# Autodesk Inventor assembly: RobotAsem
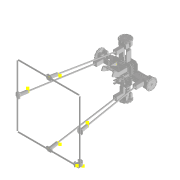
[picture p0: Inventor's stored thumbnail of the model, 180x180]
Saved by Autodesk Inventor 2022 (Build 260153000, 153)
## iProperties
Created: 2022-10-20
Part Number: RobotAsem
Document SubType Name: Assembly
Designer: MVeszpremi
Author: MVeszpremi
## Documents named in this file (20)
- C:\Users\veszp\Dropbox\180DAB CAD\RobotAsem_v2.iam
- C:\Users\veszp\Dropbox\180DAB CAD\RobotBase.ipt
- C:\Users\veszp\Dropbox\180DAB CAD\StepperMotorHolder.ipt
- C:\Users\veszp\Dropbox\180DAB CAD\RobotBaseMotorExt.ipt
- C:\Users\veszp\Dropbox\180DAB CAD\Placeholde_stepperdriverr.ipt
- C:\Users\veszp\Dropbox\180DAB CAD\Wheel.ipt
- C:\Users\veszp\Dropbox\180DAB CAD\RobotBaseMotorExtUpper.ipt
- C:\Users\veszp\Dropbox\180DAB CAD\RaspberryMount.ipt
- C:\Users\veszp\Dropbox\180DAB CAD\RaspberryPiZeroW.ipt
- C:\Users\veszp\Dropbox\180DAB CAD\BatteryMount.ipt
- C:\Users\veszp\Dropbox\180DAB CAD\ExtConnector.ipt
- C:\Users\veszp\Dropbox\180DAB CAD\DriverHolderInside_V2.ipt
- C:\Users\veszp\Dropbox\180DAB CAD\TrayHolder\Shaft_Mount_Lower.ipt
- C:\Users\veszp\Dropbox\180DAB CAD\TrayHolder\Shaft_1.ipt
- C:\Users\veszp\Dropbox\180DAB CAD\TrayHolder\Shaft_Connector_Top.ipt
- C:\Users\veszp\Dropbox\180DAB CAD\TrayHolder\Shaft_2.ipt
- C:\Users\veszp\Dropbox\180DAB CAD\TrayHolder\Shaft_Connector_Top_Corner.ipt
- C:\Users\veszp\Dropbox\180DAB CAD\StereoVisionHolder.iam
- C:\Users\veszp\Dropbox\180DAB CAD\EStopHolder.ipt
- C:\Users\veszp\Dropbox\180DAB CAD\BatteryHolder.ipt
## Components (45 placed, 19 different names)
1. RobotBase:1 — Mate:1, Mate:2, Mate:3, Mate:4, Mate:5, Mate:6, Mate:7, Mate:8, Mate:9, Mate:10, Mate:11, Mate:12, Mate:60, Mate:61, Mate:64, Mate:65, Mate:66
2. RobotBaseMotorExt:1 — Mate:1, Mate:2, Mate:3, Mate:25, Mate:26, Mate:36, Mate:37, Mate:38
3. RobotBaseMotorExt:2 — Mate:4, Mate:5, Mate:6, Mate:27, Mate:28, Mate:29
4. RobotBaseMotorExt:3 — Mate:7, Mate:8, Mate:9, Mate:33, Mate:34, Mate:35, Mate:67
5. RobotBaseMotorExt:4 — Mate:10, Mate:11, Mate:12, Mate:30, Mate:31, Mate:32
6. Placeholde_stepperdriverr:1 — Mate:25, Mate:26
7. StepperMotorHolder:1 — Mate:27, Mate:28, Mate:29, Mate:43
8. StepperMotorHolder:2 — Mate:30, Mate:31, Mate:32, Mate:41, Mate:47, Mate:48, Mate:49
9. StepperMotorHolder:3 — Mate:33, Mate:34, Mate:35, Mate:42, Mate:56
10. StepperMotorHolder:4 — Mate:36, Mate:37, Mate:38, Mate:39, Mate:40
11. Wheel:1 — Mate:39, Mate:40
12. Wheel:2 — Mate:41
13. Wheel:3 — Mate:42, Mate:67
14. Wheel:4 — Mate:43
15. RobotBaseMotorExtUpper:1 — Mate:44, Mate:45, Mate:46, Mate:47, Mate:48, Mate:49, Mate:84, Mate:85, Mate:86
16. RobotBase:2 — Mate:44, Mate:45, Mate:46, Mate:50, Mate:51, Mate:52, Mate:53, Mate:54, Mate:55, Mate:57, Mate:58, Mate:59, Mate:72, Mate:73, Mate:74, Mate:75, Mate:76, Mate:77, Mate:112, Mate:113, Mate:114
17. RobotBaseMotorExtUpper:2 — Mate:50, Mate:51, Mate:52, Mate:81, Mate:82, Mate:83, Mate:115, Mate:116
18. RobotBaseMotorExtUpper:3 — Mate:53, Mate:54, Mate:55, Mate:78, Mate:79, Mate:80, Mate:117, Mate:118, Mate:119
19. RobotBaseMotorExtUpper:4 — Mate:56, Mate:57, Mate:58, Mate:68, Mate:69, Mate:70, Mate:87, Mate:88, Mate:89
20. RaspberryMount:1 — Mate:59, Mate:60, Mate:61, Mate:62, Angle:1, Mate:63
21. RaspberryPiZeroW:1 — Mate:62, Angle:1, Mate:63
22. BatteryMount:1 — Mate:64, Mate:65, Mate:66
23. ExtConnector:1 — Mate:68, Mate:69, Mate:70
24. DriverHolderInside_V2:1 — Mate:72, Mate:73, Mate:74
25. DriverHolderInside_V2:2 — Mate:75, Mate:76, Mate:77
26. Shaft_Mount_Lower:1 — Mate:78, Mate:79, Mate:80, Mate:94, Mate:95
27. Shaft_Mount_Lower:2 — Mate:81, Mate:82, Mate:83, Mate:96, Mate:97
28. Shaft_Mount_Lower:3 — Mate:84, Mate:85, Mate:86, Mate:92, Mate:93
29. Shaft_Mount_Lower:4 — Mate:87, Mate:88, Mate:89, Mate:90, Mate:91
30. Shaft_1:1 — Mate:92, Mate:93, Mate:98, Mate:99
31. Shaft_1:2 — Mate:94, Mate:95, Mate:102, Mate:103
32. Shaft_1:3 — Mate:96, Mate:97, Mate:104, Mate:105
33. Shaft_1:4 — Mate:90, Mate:91, Mate:100, Mate:101
34. Shaft_Connector_Top:1 — Mate:98, Mate:99, Angle:3, Mate:106
35. Shaft_Connector_Top:2 — Mate:100, Mate:101, Angle:2, Mate:109
36. Shaft_Connector_Top:3 — Mate:102, Mate:103, Angle:3, Mate:107
37. Shaft_Connector_Top:4 — Mate:104, Mate:105, Angle:2, Mate:108
38. Shaft_2:1 — Mate:106
39. Shaft_2:2 — Mate:109, Mate:111
40. Shaft_2:3 — Mate:108
41. Shaft_2:4 — Mate:107, Mate:110
42. Shaft_Connector_Top_Corner:1 — Mate:110, Mate:111
43. StereoVisionHolder:1 [sub-assembly] — Mate:112, Mate:113, Mate:114
44. EStopHolder:1 — Mate:115, Mate:116
45. BatteryHolder:1 — Mate:117, Mate:118, Mate:119
## Relationships (109: Mate 106, Angle 3)
- Mate:1: RobotBase:1 ↔ RobotBaseMotorExt:1
- Mate:2: RobotBase:1 ↔ RobotBaseMotorExt:1
- Mate:3: RobotBase:1 ↔ RobotBaseMotorExt:1
- Mate:4: RobotBase:1 ↔ RobotBaseMotorExt:2
- Mate:5: RobotBase:1 ↔ RobotBaseMotorExt:2
- Mate:6: RobotBase:1 ↔ RobotBaseMotorExt:2
- Mate:7: RobotBase:1 ↔ RobotBaseMotorExt:3
- Mate:8: RobotBase:1 ↔ RobotBaseMotorExt:3
- Mate:9: RobotBase:1 ↔ RobotBaseMotorExt:3
- Mate:10: RobotBase:1 ↔ RobotBaseMotorExt:4
- Mate:11: RobotBase:1 ↔ RobotBaseMotorExt:4
- Mate:12: RobotBase:1 ↔ RobotBaseMotorExt:4
- Mate:25: RobotBaseMotorExt:1 ↔ Placeholde_stepperdriverr:1
- Mate:26 (6.5 mm): RobotBaseMotorExt:1 ↔ Placeholde_stepperdriverr:1
- Mate:27: RobotBaseMotorExt:2 ↔ StepperMotorHolder:1
- Mate:28: RobotBaseMotorExt:2 ↔ StepperMotorHolder:1
- Mate:29: RobotBaseMotorExt:2 ↔ StepperMotorHolder:1
- Mate:30: RobotBaseMotorExt:4 ↔ StepperMotorHolder:2
- Mate:31: RobotBaseMotorExt:4 ↔ StepperMotorHolder:2
- Mate:32: RobotBaseMotorExt:4 ↔ StepperMotorHolder:2
- Mate:33: RobotBaseMotorExt:3 ↔ StepperMotorHolder:3
- Mate:34: RobotBaseMotorExt:3 ↔ StepperMotorHolder:3
- Mate:35: RobotBaseMotorExt:3 ↔ StepperMotorHolder:3
- Mate:36: RobotBaseMotorExt:1 ↔ StepperMotorHolder:4
- Mate:37: RobotBaseMotorExt:1 ↔ StepperMotorHolder:4
- Mate:38: RobotBaseMotorExt:1 ↔ StepperMotorHolder:4
- Mate:39: StepperMotorHolder:4 ↔ Wheel:1
- Mate:40 (5.5 mm): StepperMotorHolder:4 ↔ Wheel:1
- Mate:41: StepperMotorHolder:2 ↔ Wheel:2
- Mate:42: StepperMotorHolder:3 ↔ Wheel:3
- Mate:43: StepperMotorHolder:1 ↔ Wheel:4
- Mate:44: RobotBaseMotorExtUpper:1 ↔ RobotBase:2
- Mate:45: RobotBaseMotorExtUpper:1 ↔ RobotBase:2
- Mate:46: RobotBaseMotorExtUpper:1 ↔ RobotBase:2
- Mate:47: StepperMotorHolder:2 ↔ RobotBaseMotorExtUpper:1
- Mate:48: StepperMotorHolder:2 ↔ RobotBaseMotorExtUpper:1
- Mate:49: StepperMotorHolder:2 ↔ RobotBaseMotorExtUpper:1
- Mate:50: RobotBase:2 ↔ RobotBaseMotorExtUpper:2
- Mate:51: RobotBase:2 ↔ RobotBaseMotorExtUpper:2
- Mate:52: RobotBase:2 ↔ RobotBaseMotorExtUpper:2
- Mate:53: RobotBase:2 ↔ RobotBaseMotorExtUpper:3
- Mate:54: RobotBase:2 ↔ RobotBaseMotorExtUpper:3
- Mate:55: RobotBase:2 ↔ RobotBaseMotorExtUpper:3
- Mate:56: StepperMotorHolder:3 ↔ RobotBaseMotorExtUpper:4
- Mate:57: RobotBase:2 ↔ RobotBaseMotorExtUpper:4
- Mate:58: RobotBase:2 ↔ RobotBaseMotorExtUpper:4
- Mate:59: RobotBase:2 ↔ RaspberryMount:1
- Mate:60: RobotBase:1 ↔ RaspberryMount:1
- Mate:61: RobotBase:1 ↔ RaspberryMount:1
- Mate:62: RaspberryMount:1 ↔ RaspberryPiZeroW:1
- Angle:1 (0 deg): RaspberryMount:1 ↔ RaspberryPiZeroW:1
- Mate:63: RaspberryMount:1 ↔ RaspberryPiZeroW:1
- Mate:64: RobotBase:1 ↔ BatteryMount:1
- Mate:65: RobotBase:1 ↔ BatteryMount:1
- Mate:66: RobotBase:1 ↔ BatteryMount:1
- Mate:67 (7.5 mm): RobotBaseMotorExt:3 ↔ Wheel:3
- Mate:68: RobotBaseMotorExtUpper:4 ↔ ExtConnector:1
- Mate:69: RobotBaseMotorExtUpper:4 ↔ ExtConnector:1
- Mate:70: RobotBaseMotorExtUpper:4 ↔ ExtConnector:1
- Mate:72: RobotBase:2 ↔ DriverHolderInside_V2:1
- Mate:73: RobotBase:2 ↔ DriverHolderInside_V2:1
- Mate:74: RobotBase:2 ↔ DriverHolderInside_V2:1
- Mate:75: RobotBase:2 ↔ DriverHolderInside_V2:2
- Mate:76: RobotBase:2 ↔ DriverHolderInside_V2:2
- Mate:77: RobotBase:2 ↔ DriverHolderInside_V2:2
- Mate:78: RobotBaseMotorExtUpper:3 ↔ Shaft_Mount_Lower:1
- Mate:79: RobotBaseMotorExtUpper:3 ↔ Shaft_Mount_Lower:1
- Mate:80: RobotBaseMotorExtUpper:3 ↔ Shaft_Mount_Lower:1
- Mate:81: RobotBaseMotorExtUpper:2 ↔ Shaft_Mount_Lower:2
- Mate:82: RobotBaseMotorExtUpper:2 ↔ Shaft_Mount_Lower:2
- Mate:83: RobotBaseMotorExtUpper:2 ↔ Shaft_Mount_Lower:2
- Mate:84: RobotBaseMotorExtUpper:1 ↔ Shaft_Mount_Lower:3
- Mate:85: RobotBaseMotorExtUpper:1 ↔ Shaft_Mount_Lower:3
- Mate:86: RobotBaseMotorExtUpper:1 ↔ Shaft_Mount_Lower:3
- Mate:87: RobotBaseMotorExtUpper:4 ↔ Shaft_Mount_Lower:4
- Mate:88: RobotBaseMotorExtUpper:4 ↔ Shaft_Mount_Lower:4
- Mate:89: RobotBaseMotorExtUpper:4 ↔ Shaft_Mount_Lower:4
- Mate:90: Shaft_Mount_Lower:4 ↔ Shaft_1:4
- Mate:91: Shaft_Mount_Lower:4 ↔ Shaft_1:4
- Mate:92: Shaft_Mount_Lower:3 ↔ Shaft_1:1
- Mate:93: Shaft_Mount_Lower:3 ↔ Shaft_1:1
- Mate:94: Shaft_Mount_Lower:1 ↔ Shaft_1:2
- Mate:95: Shaft_Mount_Lower:1 ↔ Shaft_1:2
- Mate:96: Shaft_Mount_Lower:2 ↔ Shaft_1:3
- Mate:97: Shaft_Mount_Lower:2 ↔ Shaft_1:3
- Mate:98: Shaft_1:1 ↔ Shaft_Connector_Top:1
- Mate:99: Shaft_1:1 ↔ Shaft_Connector_Top:1
- Mate:100: Shaft_1:4 ↔ Shaft_Connector_Top:2
- Mate:101: Shaft_1:4 ↔ Shaft_Connector_Top:2
- Mate:102: Shaft_1:2 ↔ Shaft_Connector_Top:3
- Mate:103: Shaft_1:2 ↔ Shaft_Connector_Top:3
- Mate:104: Shaft_1:3 ↔ Shaft_Connector_Top:4
- Mate:105: Shaft_1:3 ↔ Shaft_Connector_Top:4
- Angle:2 (0 deg): Shaft_Connector_Top:2 ↔ Shaft_Connector_Top:4
- Angle:3 (0 deg): Shaft_Connector_Top:1 ↔ Shaft_Connector_Top:3
- Mate:106: Shaft_Connector_Top:1 ↔ Shaft_2:1
- Mate:107: Shaft_Connector_Top:3 ↔ Shaft_2:4
- Mate:108: Shaft_Connector_Top:4 ↔ Shaft_2:3
- Mate:109: Shaft_Connector_Top:2 ↔ Shaft_2:2
- Mate:110: Shaft_2:4 ↔ Shaft_Connector_Top_Corner:1
- Mate:111: Shaft_2:2 ↔ Shaft_Connector_Top_Corner:1
- Mate:112: RobotBase:2 ↔ StereoVisionHolder:1
- Mate:113: RobotBase:2 ↔ StereoVisionHolder:1
- Mate:114: RobotBase:2 ↔ StereoVisionHolder:1
- Mate:115: RobotBaseMotorExtUpper:2 ↔ EStopHolder:1
- Mate:116: RobotBaseMotorExtUpper:2 ↔ EStopHolder:1
- Mate:117: RobotBaseMotorExtUpper:3 ↔ BatteryHolder:1
- Mate:118: RobotBaseMotorExtUpper:3 ↔ BatteryHolder:1
- Mate:119: RobotBaseMotorExtUpper:3 ↔ BatteryHolder:1
